# Autodesk Inventor assembly: Frame
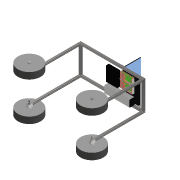
[picture p0: Inventor's stored thumbnail of the model, 180x180]
Saved by Autodesk Inventor 2022 (Build 260153000, 153)
## iProperties
_SolveAssemblyDoc: Frame Generator Solve Assembly
_Version: 25.0.0
Created: 2024-04-01
Part Number: Frame
Document SubType Name: Assembly
Designer: LaptopJR
Author: LaptopJR
## Documents named in this file (17)
- C:\Users\LaptopJR\Documents\Ideation AI\EcoTerrabot\Chassis\CAD files\Mock platform\Frame.iam
- C:\Users\LaptopJR\Documents\Ideation AI\EcoTerrabot\Chassis\CAD files\Frame.ipt
- C:\Users\LaptopJR\Documents\Ideation AI\EcoTerrabot\Chassis\CAD files\Mock platform\Frame\Frame\Frame 1711976507957.iam
- C:\Users\LaptopJR\Documents\Ideation AI\EcoTerrabot\Chassis\CAD files\Mock platform\Bearing holder.ipt
- C:\Users\LaptopJR\Documents\Ideation AI\EcoTerrabot\Chassis\CAD files\Mock platform\Bearing 6204-2RSH\skf_bearing_6204-2rsh_2.iam
- C:\Users\LaptopJR\Documents\Ideation AI\EcoTerrabot\Chassis\CAD files\Wheel 350x100x20.ipt
- C:\Users\LaptopJR\Documents\Inventor\Content Center Files\R2022\en-US\ANSI B18.2.3.6M\ANSI B18.2.3.6M - M20 x 2.5 x 200.ipt
- C:\Users\LaptopJR\Documents\Inventor\Content Center Files\R2022\en-US\ANSI B18.2.4.6M\ANSI B18.2.4.6M - M20 x 2.5 - 0.ipt
- C:\Users\LaptopJR\Documents\Ideation AI\EcoTerrabot\Chassis\CAD files\Mock platform\Bearing holder_MIR.ipt
- C:\Users\LaptopJR\Documents\Ideation AI\EcoTerrabot\Chassis\CAD files\Mock platform\Bearing 6204-2RSH\skf_bearing_6204-2rsh_2_MIR.iam
- C:\Users\LaptopJR\Documents\Ideation AI\EcoTerrabot\Chassis\CAD files\Wheel 350x100x20_MIR.ipt
- C:\Users\LaptopJR\Documents\Ideation AI\EcoTerrabot\Chassis\CAD files\Mock platform\Battery_Greencell_EBIKE12STD_11Ah.ipt
- C:\Users\LaptopJR\Documents\Ideation AI\EcoTerrabot\Chassis\CAD files\SD-100\SD-100.iam
- C:\Users\LaptopJR\Documents\Ideation AI\EcoTerrabot\Chassis\CAD files\Mock platform\SCANLAB-SNZ0045937.ipt
- C:\Users\LaptopJR\Documents\Ideation AI\EcoTerrabot\Chassis\CAD files\Mock platform\Laptop_MSI_KATANA_GF76_11UG.ipt
- C:\Users\LaptopJR\Documents\Ideation AI\EcoTerrabot\Chassis\CAD files\Mock platform\Laptop-ecke.ipt
- C:\Users\LaptopJR\Documents\Ideation AI\EcoTerrabot\Chassis\CAD files\Mock platform\Laptop-ecke-l.ipt
## Components (30 placed, 16 different names)
1. Frame:1 — Mate:3
2. Frame 1711976507957:1 [sub-assembly] — Mate:3, Mate:4, Mate:5, Flush:1, Mate:11, Flush:2, Mate:13, Flush:3, Mate:14, Mate:15, Mate:16, Flush:6, Mate:17, Flush:7, Mate:18, Flush:8, Mate:19, Flush:9
3. Bearing holder_MIR:1
4. skf_bearing_6204-2rsh_2_MIR:1 [sub-assembly]
5. Wheel 350x100x20_MIR:1
6. Heavy Hex Bolt - Metric M20 x 2.5 x 200:3
7. Heavy Hex Nut Metric M20 x 2.5:3
8. Bearing holder_MIR:2
9. skf_bearing_6204-2rsh_2_MIR:2 [sub-assembly]
10. Wheel 350x100x20_MIR:2
11. Heavy Hex Bolt - Metric M20 x 2.5 x 200:4
12. Heavy Hex Nut Metric M20 x 2.5:4
13. Battery_Greencell_EBIKE12STD_11Ah:1 — Mate:13, Flush:3
14. SD-100:1 [sub-assembly] — Flush:4, Flush:5
15. SD-100:2 [sub-assembly] — Mate:14, Flush:4, Flush:5
16. SCANLAB-SNZ0045937:1 — Mate:15
17. Laptop_MSI_KATANA_GF76_11UG:1 — Mate:16, Flush:6
18. Laptop-ecke:1 — Mate:17, Flush:7
19. Laptop-ecke:2 — Mate:18, Flush:8
20. Laptop-ecke-l:1 — Mate:19, Flush:9
21. Bearing holder:1 — Mate:4, Mate:5, Flush:1, Mate:6, Mate:7
22. skf_bearing_6204-2rsh_2:1 [sub-assembly] — Mate:6, Mate:7, Mate:8, Mate:12
23. Wheel 350x100x20:1 — Insert:1, Mate:12
24. Heavy Hex Bolt - Metric M20 x 2.5 x 200:1 — Insert:1, Mate:8, Mate:10
25. Heavy Hex Nut Metric M20 x 2.5:1 — Mate:10, Mate:11
26. Bearing holder:2
27. skf_bearing_6204-2rsh_2:2 [sub-assembly]
28. Wheel 350x100x20:2
29. Heavy Hex Bolt - Metric M20 x 2.5 x 200:2
30. Heavy Hex Nut Metric M20 x 2.5:2
## Component patterns: (2 elements, first: Bearing holder:1 + skf_bearing_6204-2rsh_2:1 + Wheel 350x100x20:1 + Heavy Hex Bolt - Metric M20 x 2.5 x 200:1 + Heavy Hex Nut Metric M20 x 2.5:1)
## Relationships (26: Mate 16, Flush 9, Insert 1)
- Mate:3: Frame:1 ↔ Frame 1711976507957:1
- Mate:4: Frame 1711976507957:1 ↔ Bearing holder:1
- Mate:5: Frame 1711976507957:1 ↔ Bearing holder:1
- Flush:1: Frame 1711976507957:1 ↔ Bearing holder:1
- Mate:6: Bearing holder:1 ↔ skf_bearing_6204-2rsh_2:1
- Mate:7: Bearing holder:1 ↔ skf_bearing_6204-2rsh_2:1
- Insert:1: Wheel 350x100x20:1 ↔ Heavy Hex Bolt - Metric M20 x 2.5 x 200:1
- Mate:8: skf_bearing_6204-2rsh_2:1 ↔ Heavy Hex Bolt - Metric M20 x 2.5 x 200:1
- Mate:10: Heavy Hex Bolt - Metric M20 x 2.5 x 200:1 ↔ Heavy Hex Nut Metric M20 x 2.5:1
- Mate:11: Frame 1711976507957:1 ↔ Heavy Hex Nut Metric M20 x 2.5:1
- Mate:12: skf_bearing_6204-2rsh_2:1 ↔ Wheel 350x100x20:1
- Flush:2 (-230 mm): Frame 1711976507957:1
- Mate:13: Frame 1711976507957:1 ↔ Battery_Greencell_EBIKE12STD_11Ah:1
- Flush:3 (300 mm): Frame 1711976507957:1 ↔ Battery_Greencell_EBIKE12STD_11Ah:1
- Mate:14: Frame 1711976507957:1 ↔ SD-100:2
- Flush:4: SD-100:1 ↔ SD-100:2
- Flush:5: SD-100:1 ↔ SD-100:2
- Mate:15 (5 mm): Frame 1711976507957:1 ↔ SCANLAB-SNZ0045937:1
- Mate:16 (4 mm): Frame 1711976507957:1 ↔ Laptop_MSI_KATANA_GF76_11UG:1
- Flush:6 (31 mm): Frame 1711976507957:1 ↔ Laptop_MSI_KATANA_GF76_11UG:1
- Mate:17: Frame 1711976507957:1 ↔ Laptop-ecke:1
- Flush:7: Frame 1711976507957:1 ↔ Laptop-ecke:1
- Mate:18: Frame 1711976507957:1 ↔ Laptop-ecke:2
- Flush:8: Frame 1711976507957:1 ↔ Laptop-ecke:2
- Mate:19: Frame 1711976507957:1 ↔ Laptop-ecke-l:1
- Flush:9: Frame 1711976507957:1 ↔ Laptop-ecke-l:1
